# Autodesk Inventor assembly: Assembly
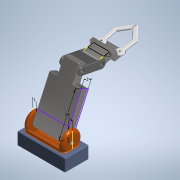
[picture p0: Inventor's stored thumbnail of the model, 180x180]
Saved by Autodesk Inventor 2022 (Build 260153000, 153)
## iProperties
Part Number: Assembly
Document SubType Name: Assembly
Designer: Suhas Gopal
Author: suhas
## Documents named in this file (6)
- D:\Projects\Playground\robotic-arm\Assemblies\Assembly.iam
- D:\Projects\Playground\robotic-arm\Parts\Base.ipt
- D:\Projects\Playground\robotic-arm\Parts\Link1.ipt
- D:\Projects\Playground\robotic-arm\Parts\Link2.ipt
- D:\Projects\Playground\robotic-arm\Parts\Link3.ipt
- D:\Projects\Playground\robotic-arm\Parts\Gripper.ipt
## Components (6 placed, 5 different names)
1. Base:1 — Rotational:1, Mate:3
2. Link1:1 — Rotational:1, Rotational:2, Mate:2, Mate:3
3. Link2:1 — Rotational:2, Rotational:3, Mate:1, Mate:2
4. Link3:1 — Rotational:3, Mate:1, Rotational:5, Rotational:6
5. Gripper:1 — Rotational:5
6. Gripper:2 — Rotational:6
## Relationships (8: RevoluteJoint 5, Mate 3)
- Rotational:1 [RevoluteJoint] (-40.5 mm): Base:1 ↔ Link1:1
- Rotational:2 [RevoluteJoint] (21.75 mm): Link1:1 ↔ Link2:1
- Rotational:3 [RevoluteJoint] (20.25 mm): Link2:1 ↔ Link3:1
- Mate:1: Link2:1 ↔ Link3:1
- Mate:2: Link1:1 ↔ Link2:1
- Mate:3: Base:1 ↔ Link1:1
- Rotational:5 [RevoluteJoint] (-3.5 mm): Link3:1 ↔ Gripper:1
- Rotational:6 [RevoluteJoint] (-3.5 mm): Link3:1 ↔ Gripper:2
